# Autodesk Inventor assembly: Naroznik
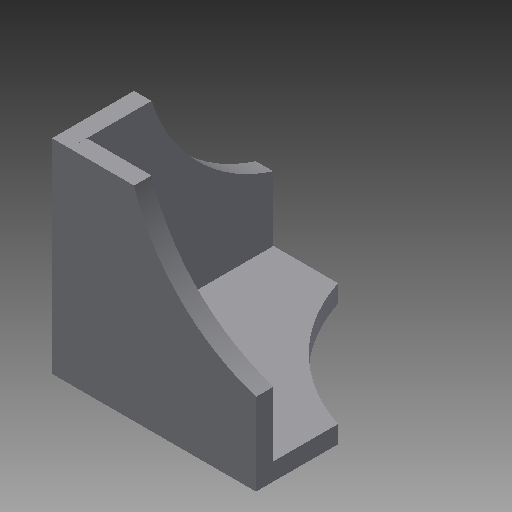
[picture p0: Inventor's stored thumbnail of the model, 512x512]
Saved by Autodesk Inventor 2018 (Build 220112000, 112)
## iProperties
Created: 2018-10-22
Part Number: Naroznik
Material: Ogólny
Document SubType Name: Assembly
Designer: EWA
Author: EWA
## Documents named in this file (4)
- C:\Users\EWA\Documents\Inventor\Kostka\Naroznik.iam
- C:\Users\EWA\Documents\Inventor\Kostka\Naroznik_54x54.ipt
- C:\Users\EWA\Documents\Inventor\Kostka\Naroznik_60x54.ipt
- C:\Users\EWA\Documents\Inventor\Kostka\Naroznik_60x60.ipt
## Components (3 placed, 3 different names)
1. Naroznik_54x54:1 — Zestawiający:2, Zestawiający:3, Równoległy:3
2. Naroznik_60x54:1 — Zestawiający:1, Równoległy:1, Równoległy:2, Zestawiający:2
3. Naroznik_60x60:1 — Zestawiający:1, Równoległy:1, Równoległy:2, Zestawiający:3, Równoległy:3
## Relationships (6: Mate 3, Flush 3)
- Zestawiający:1 [Mate]: Naroznik_60x54:1 ↔ Naroznik_60x60:1
- Równoległy:1 [Flush]: Naroznik_60x54:1 ↔ Naroznik_60x60:1
- Równoległy:2 [Flush]: Naroznik_60x54:1 ↔ Naroznik_60x60:1
- Zestawiający:2 [Mate]: Naroznik_54x54:1 ↔ Naroznik_60x54:1
- Zestawiający:3 [Mate]: Naroznik_54x54:1 ↔ Naroznik_60x60:1
- Równoległy:3 [Flush]: Naroznik_54x54:1 ↔ Naroznik_60x60:1
